# Autodesk Inventor assembly: Claw2017-18
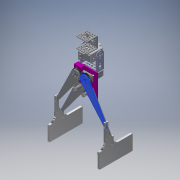
[picture p0: Inventor's stored thumbnail of the model, 180x180]
Saved by Autodesk Inventor 2017 (Build 210142000, 142)
## iProperties
Created: 2017-09-28
Part Number: Claw2017-18
Document SubType Name: Assembly
Designer: User
Author: User
## Documents named in this file (12)
- C:\Robotics\CAD\2017-18_CAD\Claw2017-18.iam
- C:\Robotics\CAD\2017-18_CAD\Miscellaneous\ClawServoHolder.ipt
- C:\Robotics\CAD\COTSParts\Tetrix\Tetrix Gear 40T.ipt
- C:\Robotics\CAD\2017-18_CAD\Miscellaneous\ClawLinkage.ipt
- C:\Robotics\CAD\COTSParts\Vex\91259A576_ALLOY STEEL SHOULDER SCREW.ipt
- C:\Robotics\CAD\COTSParts\Vex\91259A581_ALLOY STEEL SHOULDER SCREW.ipt
- C:\Robotics\CAD\2017-18_CAD\Miscellaneous\ClawSpacer.ipt
- C:\Robotics\CAD\COTSParts\Tetrix\Tetrix bracket - single servo.ipt
- C:\Robotics\CAD\2017-18_CAD\Miscellaneous\TheClaw.iam
- C:\Robotics\CAD\2017-18_CAD\Miscellaneous\2BarClawPaddle2.0.ipt
- C:\Robotics\CAD\COTSParts\Rev\REV-41-1097.iam
- C:\Robotics\CAD\COTSParts\Actobotics\585 parts\585440.ipt
## Components (18 placed, 11 different names)
1. ClawServoHolder:1 — Mate:11, Mate:12, Mate:43, Mate:44, Mate:45, Mate:46, Mate:53, Mate:54, Mate:58, Insert:1, Angle:1, Angle:2
2. Tetrix Gear 40T:1 — Flush:5, Mate:19, Mate:91
3. Tetrix Gear 40T:2 — Mate:11, Mate:12, Flush:5, Mate:23
4. ClawLinkage:1 — Mate:19, Mate:84, Mate:86, Mate:92, Rotation:1
5. ClawLinkage:2 — Mate:23, Mate:87, Mate:93, Rotation:1
6. 91259A576_ALLOY STEEL SHOULDER SCREW:1 — Mate:43, Mate:44, Flush:6, Flush:7, Mate:93
7. 91259A581_ALLOY STEEL SHOULDER SCREW:3 — Mate:45, Flush:6, Mate:47, Mate:52
8. 91259A581_ALLOY STEEL SHOULDER SCREW:4 — Mate:46, Flush:7, Mate:49, Mate:51
9. ClawLinkage:3 — Mate:47, Flush:8, Mate:85
10. ClawLinkage:4 — Mate:49, Mate:58, Flush:8, Mate:88, Mate:89
11. ClawSpacer:1 — Mate:51, Mate:53
12. ClawSpacer:2 — Mate:52, Mate:54
13. Tetrix bracket - single servo:1 — Insert:2, Angle:2, Mate:90, Angle:3, Insert:3
14. TheClaw:1 [sub-assembly] — Mate:90, Angle:3, Insert:3, Insert:4, Angle:4
15. 2BarClawPaddle2.0:1 — Mate:87, Mate:88, Mate:89
16. 2BarClawPaddle2.0:2 — Mate:84, Mate:85, Mate:86
17. REV-41-1097:1 [sub-assembly] — Insert:1, Angle:1, Insert:2, Mate:91, Mate:92
18. 585440:1 — Insert:4, Angle:4
## Relationships (38: Mate 25, Flush 4, Insert 4, Angle 4, RelateRotation 1)
- Mate:11: ClawServoHolder:1 ↔ Tetrix Gear 40T:2
- Mate:12: ClawServoHolder:1 ↔ Tetrix Gear 40T:2
- Flush:5: Tetrix Gear 40T:1 ↔ Tetrix Gear 40T:2
- Mate:19: Tetrix Gear 40T:1 ↔ ClawLinkage:1
- Mate:23: Tetrix Gear 40T:2 ↔ ClawLinkage:2
- Mate:43: ClawServoHolder:1 ↔ 91259A576_ALLOY STEEL SHOULDER SCREW:1
- Mate:44: ClawServoHolder:1 ↔ 91259A576_ALLOY STEEL SHOULDER SCREW:1
- Mate:45: ClawServoHolder:1 ↔ 91259A581_ALLOY STEEL SHOULDER SCREW:3
- Flush:6: 91259A576_ALLOY STEEL SHOULDER SCREW:1 ↔ 91259A581_ALLOY STEEL SHOULDER SCREW:3
- Mate:46: ClawServoHolder:1 ↔ 91259A581_ALLOY STEEL SHOULDER SCREW:4
- Flush:7: 91259A576_ALLOY STEEL SHOULDER SCREW:1 ↔ 91259A581_ALLOY STEEL SHOULDER SCREW:4
- Mate:47: 91259A581_ALLOY STEEL SHOULDER SCREW:3 ↔ ClawLinkage:3
- Mate:49: 91259A581_ALLOY STEEL SHOULDER SCREW:4 ↔ ClawLinkage:4
- Mate:51: 91259A581_ALLOY STEEL SHOULDER SCREW:4 ↔ ClawSpacer:1
- Mate:52: 91259A581_ALLOY STEEL SHOULDER SCREW:3 ↔ ClawSpacer:2
- Mate:53: ClawServoHolder:1 ↔ ClawSpacer:1
- Mate:54: ClawServoHolder:1 ↔ ClawSpacer:2
- Mate:58: ClawServoHolder:1 ↔ ClawLinkage:4
- Flush:8: ClawLinkage:3 ↔ ClawLinkage:4
- Mate:84: ClawLinkage:1 ↔ 2BarClawPaddle2.0:2
- Mate:85: ClawLinkage:3 ↔ 2BarClawPaddle2.0:2
- Mate:86: ClawLinkage:1 ↔ 2BarClawPaddle2.0:2
- Mate:87: ClawLinkage:2 ↔ 2BarClawPaddle2.0:1
- Mate:88: ClawLinkage:4 ↔ 2BarClawPaddle2.0:1
- Mate:89: ClawLinkage:4 ↔ 2BarClawPaddle2.0:1
- Insert:1: ClawServoHolder:1 ↔ REV-41-1097:1
- Angle:1 (270 deg): ClawServoHolder:1 ↔ REV-41-1097:1
- Insert:2 (2.667 mm): Tetrix bracket - single servo:1 ↔ REV-41-1097:1
- Angle:2 (0 deg): ClawServoHolder:1 ↔ Tetrix bracket - single servo:1
- Mate:90: Tetrix bracket - single servo:1 ↔ TheClaw:1
- Angle:3 (0 deg): Tetrix bracket - single servo:1 ↔ TheClaw:1
- Insert:3: Tetrix bracket - single servo:1 ↔ TheClaw:1
- Mate:91: Tetrix Gear 40T:1 ↔ REV-41-1097:1
- Mate:92: ClawLinkage:1 ↔ REV-41-1097:1
- Mate:93: ClawLinkage:2 ↔ 91259A576_ALLOY STEEL SHOULDER SCREW:1
- Rotation:1 [RelateRotation] (1 ul): ClawLinkage:1 ↔ ClawLinkage:2
- Insert:4: TheClaw:1 ↔ 585440:1
- Angle:4 (0 deg): TheClaw:1 ↔ 585440:1
